# Autodesk Inventor assembly: chassis-weld
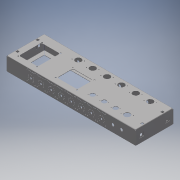
[picture p0: Inventor's stored thumbnail of the model, 180x180]
Saved by Autodesk Inventor 2016 (Build 200138000, 138)
## iProperties
Created: 2015-10-28
Part Number: chassis-weld
Document SubType Name: Weldment
Designer: jeremyhale
Weld Material: Welded Aluminum-6061
Author: jeremyhale
## Documents named in this file (2)
- \\psf\Home\Documents\Poorhouse\git\p0001\chassis-weld.iam
- \\psf\Home\Documents\Poorhouse\git\p0001\chassis.ipt
## Components (1 placed, 1 different names)
1. chassis:1 — Flush:1
## Relationships (1: Flush 1)
- Flush:1: chassis:1
